# Autodesk Inventor assembly: HERA_NODE_ENCLOSURE_ASSEMBLY
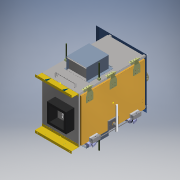
[picture p0: Inventor's stored thumbnail of the model, 180x180]
Saved by Autodesk Inventor 2018 (Build 220112000, 112)
## iProperties
Created: 2018-10-02
Part Number: HERA_NODE_ENCLOSURE_ASSEMBLY
Document SubType Name: Assembly
Designer: Francois
Mass: 169996 g
Surface Area: 258850 cm^2
Volume: 23149 cm^3
Density: 7.34355 g/cm^3
Author: Francois
## Documents named in this file (29)
- D:\ITC\DRAWINGS\SKA PROJECT\HERA NODE\HERA NODE 2018 TENDER SUBMISIONS\ASSEMBLY\HERA_NODE_ENCLOSURE_ASSEMBLY.iam
- D:\ITC\DRAWINGS\SKA PROJECT\HERA NODE\HERA NODE 2018 TENDER SUBMISIONS\PARTS\HERA_NODE_BOTTOM_PLATE.ipt
- D:\ITC\DRAWINGS\SKA PROJECT\HERA NODE\HERA NODE 2018 TENDER SUBMISIONS\PARTS\HERA_NODE_LEFT_SIDE_PLATE.ipt
- D:\ITC\DRAWINGS\SKA PROJECT\HERA NODE\HERA NODE 2018 TENDER SUBMISIONS\PARTS\HERA_NODE_RIGHT_SIDE_PLATE.ipt
- D:\ITC\DRAWINGS\SKA PROJECT\HERA NODE\HERA NODE 2018 TENDER SUBMISIONS\PARTS\HERA_NODE_TOP_PLATE.ipt
- D:\ITC\DRAWINGS\SKA PROJECT\HERA NODE\HERA NODE 2018 TENDER SUBMISIONS\PARTS\HERA_NODE_BACK_PLATE.ipt
- D:\ITC\DRAWINGS\SKA PROJECT\HERA NODE\HERA NODE 2018 TENDER SUBMISIONS\ASSEMBLY\HERA_NODE_FOOTPLATE_ASSEMBLY.iam
- D:\ITC\DRAWINGS\SKA PROJECT\HERA NODE\HERA NODE 2018 TENDER SUBMISIONS\ASSEMBLY\HERA_NODE_DOOR_ASSEMBLY.iam
- D:\ITC\DRAWINGS\SKA PROJECT\HERA NODE\HERA NODE 2018 TENDER SUBMISIONS\PARTS\FILTER PLATES\FILTER_PLATE_RP.ipt
- D:\ITC\DRAWINGS\SKA PROJECT\HERA NODE\HERA NODE 2018 TENDER SUBMISIONS\PARTS\FILTER PLATES\FILTER_PLATE_LP.ipt
- D:\ITC\DRAWINGS\SKA PROJECT\HERA NODE\HERA NODE 2018 TENDER SUBMISIONS\PARTS\HINGES\HINGE_ASSEMBLY.iam
- D:\ITC\DRAWINGS\SKA PROJECT\HERA NODE\HERA NODE 2018 TENDER SUBMISIONS\PARTS\FILTER PLATES\FILTER_PANEL_COVER_RP.ipt
- D:\ITC\DRAWINGS\SKA PROJECT\HERA NODE\HERA NODE 2018 TENDER SUBMISIONS\PARTS\LIFTING LUGS\LIFTING_LUG_SUPPORT.ipt
- D:\ITC\DRAWINGS\SKA PROJECT\HERA NODE\HERA NODE 2018 TENDER SUBMISIONS\PARTS\ROOF_PANEL.ipt
- D:\ITC\DRAWINGS\SKA PROJECT\HERA NODE\HERA NODE 2018 TENDER SUBMISIONS\PARTS\LIFTING LUGS\CARRY_HANDLE_SUPPORT.ipt
- D:\ITC\DRAWINGS\SKA PROJECT\HERA NODE\HERA NODE 2018 TENDER SUBMISIONS\PARTS\LIFTING LUGS\CARRY_HANDLE.ipt
- D:\ITC\DRAWINGS\SKA PROJECT\HERA NODE\HERA NODE 2018 TENDER SUBMISIONS\PARTS\DOOR HANDLE\DOOR_LOCK_CATCH.ipt
- D:\ITC\DRAWINGS\SKA PROJECT\HERA NODE\HERA NODE 2018 TENDER SUBMISIONS\ASSEMBLY\PART 1.ipt
- D:\ITC\DRAWINGS\SKA PROJECT\HERA NODE\HERA NODE 2018 TENDER SUBMISIONS\PARTS\VENTS\HERA_NODE_TOP_BOTTOM_ATTENUVENT.ipt
- D:\ITC\DRAWINGS\SKA PROJECT\HERA NODE\HERA NODE 2018 TENDER SUBMISIONS\PARTS\DINRAIL\DIN Rail (TS) 35mm Wide v1.ipt
- D:\ITC\DRAWINGS\SKA PROJECT\HERA NODE\HERA NODE 2018 TENDER SUBMISIONS\PARTS\DINRAIL\DIN Rail (TS) 35mm Wide v1\TS35x7.5 mm H - 6.2 mm dia slot - 225 mm long.ipt
- D:\ITC\DRAWINGS\SKA PROJECT\HERA NODE\HERA NODE 2018 TENDER SUBMISIONS\PARTS\LIFTING LUGS\M10 EYEBOLT.ipt
- D:\ITC\DRAWINGS\SKA PROJECT\HERA NODE\HERA NODE 2018 TENDER SUBMISIONS\PARTS\ALLBRO DB BOX\ALBRO_DB_BOX.iam
- D:\ITC\DRAWINGS\INVENTOR LIBRARY\DOOR HANDLES\SKA EN ABSA DEUR\DOOR HANDLE.iam
- D:\ITC\DRAWINGS\SKA PROJECT\HERA NODE\HERA NODE 2018 TENDER SUBMISIONS\PARTS\16A POWER FILTER\FILTER ASSEMBLY.iam
- D:\ITC\DRAWINGS\SKA PROJECT\HERA NODE\HERA NODE 2018 TENDER SUBMISIONS\PARTS\HINGES\FILTER PLATE COVER HINGES\4-3-4 bullet hinge.ipt
- D:\ITC\DRAWINGS\SKA PROJECT\HERA NODE\HERA NODE 2018 TENDER SUBMISIONS\PARTS\U_BRACKETS.ipt
- D:\ITC\DRAWINGS\SKA PROJECT\HERA NODE\HERA NODE 2018 TENDER SUBMISIONS\PARTS\CABLE TIE DOWN BAR\CABLE_TIE_DOWN_ASSEMBLY.iam
- D:\ITC\DRAWINGS\SKA PROJECT\HERA NODE\HERA NODE 2018 TENDER SUBMISIONS\PARTS\WHIRLEY BIRD\WHIRLEY BIRD.iam
## Components (50 placed, 27 different names)
1. HERA_NODE_BOTTOM_PLATE:1 — Mate:2, Flush:3, Flush:4, Mate:4, Flush:7, Flush:8, Mate:7, Mate:8, Mate:53, Mate:55
2. HERA_NODE_LEFT_SIDE_PLATE:1 — Mate:4, Flush:7, Flush:8, Mate:6, Flush:10, Flush:11, Mate:13, Mate:14, Mate:15, Mate:27, Flush:21, Flush:23, Flush:24, Flush:30, Mate:43, Mate:44, Flush:36, Mate:66, Mate:67, Mate:68, Mate:72
3. HERA_NODE_RIGHT_SIDE_PLATE:1 — Mate:2, Flush:3, Flush:4, Mate:3, Flush:5, Flush:6, Flush:12, Flush:13, Flush:14, Mate:10, Mate:11, Mate:12, Mate:26, Flush:25, Flush:26, Flush:27, Flush:29, Mate:41, Flush:32, Mate:42, Mate:64, Mate:65, Mate:70, Mate:73
4. HERA_NODE_TOP_PLATE:1 — Mate:3, Flush:5, Flush:6, Mate:5, Flush:9, Mate:9, Flush:15, Mate:32, Mate:33, Mate:34, Mate:35, Mate:54
5. HERA_NODE_BACK_PLATE:1 — Mate:5, Mate:6, Flush:9, Flush:22, Flush:28, Flush:34, Flush:38, Mate:56, Mate:61, Mate:63
6. HERA_NODE_FOOTPLATE_ASSEMBLY:1 [sub-assembly] — Mate:7, Flush:10, Flush:11, Flush:35, Flush:37
7. HERA_NODE_FOOTPLATE_ASSEMBLY:2 [sub-assembly] — Mate:8, Flush:12, Flush:13, Flush:31, Flush:33
8. HERA_NODE_DOOR_ASSEMBLY:1 [sub-assembly] — Mate:9, Flush:14, Flush:15, Mate:22, Flush:16, Mate:23, Flush:18, Mate:24, Flush:20, Mate:62, Flush:43, Flush:44
9. FILTER_PLATE_RP:1 — Mate:10, Mate:11, Mate:12, Mate:28, Mate:29
10. FILTER_PLATE_LP:1 — Mate:13, Mate:14, Mate:15, Mate:30, Mate:31
11. HINGE_ASSEMBLY:1 [sub-assembly] — Mate:22, Flush:16, Flush:17, Flush:19, Mate:25, Flush:20
12. HINGE_ASSEMBLY:2 [sub-assembly] — Mate:23, Flush:17, Flush:18
13. HINGE_ASSEMBLY:3 [sub-assembly] — Mate:24, Flush:19, Mate:25
14. FILTER_PANEL_COVER_RP:1 — Mate:26, Mate:28, Mate:29, Flush:45, Flush:46, Mate:71, Flush:50, Flush:53
15. FILTER_PANEL_COVER_RP:2 — Mate:27, Mate:30, Mate:31, Flush:47, Flush:48, Mate:69, Flush:49, Flush:54
16. LIFTING_LUG_SUPPORT:1 — Mate:33, Flush:23, Flush:24, Mate:60
17. LIFTING_LUG_SUPPORT:2 — Mate:34, Flush:25, Flush:26, Mate:36, Mate:59
18. LIFTING_LUG_SUPPORT:3 — Mate:32, Flush:21, Flush:22, Mate:58
19. LIFTING_LUG_SUPPORT:4 — Mate:35, Flush:27, Flush:28, Mate:57
20. ROOF_PANEL:1 — Mate:36, Flush:29, Flush:30, Mate:74
21. CARRY_HANDLE_SUPPORT:1 — Mate:44, Flush:35, Flush:36, Mate:46
22. CARRY_HANDLE_SUPPORT:2 — Mate:43, Flush:37, Flush:38, Mate:45
23. CARRY_HANDLE_SUPPORT:3 — Mate:42, Flush:33, Flush:34, Mate:48
24. CARRY_HANDLE_SUPPORT:4 — Mate:41, Flush:31, Flush:32, Mate:47
25. CARRY_HANDLE:1 — Mate:48
26. CARRY_HANDLE:2 — Mate:47
27. CARRY_HANDLE:3 — Mate:45
28. CARRY_HANDLE:4 — Mate:46
29. DOOR_LOCK_CATCH:1
30. DOOR_LOCK_CATCH:2
31. PART 1:1 — Mate:53
32. HERA_NODE_TOP_BOTTOM_ATTENUVENT:1 — Mate:54
33. HERA_NODE_TOP_BOTTOM_ATTENUVENT:2 — Mate:55
34. TS35x7.5 mm H - 6.2 mm dia slot - 225 mm long:1 — Mate:56
35. M10 EYEBOLT:1 — Mate:59
36. M10 EYEBOLT:2 — Mate:57
37. M10 EYEBOLT:3 — Mate:60
38. M10 EYEBOLT:4 — Mate:58
39. ALBRO_DB_BOX:1 [sub-assembly] — Mate:61
40. DOOR HANDLE:2 [sub-assembly] — Mate:62, Flush:43, Flush:44
41. FILTER ASSEMBLY:1 [sub-assembly] — Mate:63
42. 4-3-4 bullet hinge:1 — Mate:64, Flush:45
43. 4-3-4 bullet hinge:2 — Mate:65, Flush:46
44. 4-3-4 bullet hinge:3 — Mate:66, Flush:47
45. 4-3-4 bullet hinge:4 — Mate:67, Flush:48
46. U_BRACKETS:1 — Mate:68, Mate:69, Flush:49, Flush:55
47. U_BRACKETS:2 — Mate:70, Mate:71, Flush:50, Flush:56
48. CABLE_TIE_DOWN_ASSEMBLY:1 [sub-assembly] — Mate:73, Flush:53, Flush:56
49. CABLE_TIE_DOWN_ASSEMBLY:2 [sub-assembly] — Mate:72, Flush:54, Flush:55
50. WHIRLEY BIRD:1 [sub-assembly] — Mate:74
## Relationships (107: Mate 59, Flush 48)
- Mate:2: HERA_NODE_BOTTOM_PLATE:1 ↔ HERA_NODE_RIGHT_SIDE_PLATE:1
- Flush:3: HERA_NODE_BOTTOM_PLATE:1 ↔ HERA_NODE_RIGHT_SIDE_PLATE:1
- Flush:4: HERA_NODE_BOTTOM_PLATE:1 ↔ HERA_NODE_RIGHT_SIDE_PLATE:1
- Mate:3: HERA_NODE_RIGHT_SIDE_PLATE:1 ↔ HERA_NODE_TOP_PLATE:1
- Flush:5: HERA_NODE_RIGHT_SIDE_PLATE:1 ↔ HERA_NODE_TOP_PLATE:1
- Flush:6: HERA_NODE_RIGHT_SIDE_PLATE:1 ↔ HERA_NODE_TOP_PLATE:1
- Mate:4: HERA_NODE_BOTTOM_PLATE:1 ↔ HERA_NODE_LEFT_SIDE_PLATE:1
- Flush:7: HERA_NODE_BOTTOM_PLATE:1 ↔ HERA_NODE_LEFT_SIDE_PLATE:1
- Flush:8: HERA_NODE_BOTTOM_PLATE:1 ↔ HERA_NODE_LEFT_SIDE_PLATE:1
- Mate:5: HERA_NODE_TOP_PLATE:1 ↔ HERA_NODE_BACK_PLATE:1
- Mate:6: HERA_NODE_LEFT_SIDE_PLATE:1 ↔ HERA_NODE_BACK_PLATE:1
- Flush:9: HERA_NODE_TOP_PLATE:1 ↔ HERA_NODE_BACK_PLATE:1
- Mate:7: HERA_NODE_BOTTOM_PLATE:1 ↔ HERA_NODE_FOOTPLATE_ASSEMBLY:1
- Flush:10: HERA_NODE_LEFT_SIDE_PLATE:1 ↔ HERA_NODE_FOOTPLATE_ASSEMBLY:1
- Flush:11: HERA_NODE_LEFT_SIDE_PLATE:1 ↔ HERA_NODE_FOOTPLATE_ASSEMBLY:1
- Mate:8: HERA_NODE_BOTTOM_PLATE:1 ↔ HERA_NODE_FOOTPLATE_ASSEMBLY:2
- Flush:12: HERA_NODE_RIGHT_SIDE_PLATE:1 ↔ HERA_NODE_FOOTPLATE_ASSEMBLY:2
- Flush:13: HERA_NODE_RIGHT_SIDE_PLATE:1 ↔ HERA_NODE_FOOTPLATE_ASSEMBLY:2
- Mate:9: HERA_NODE_TOP_PLATE:1 ↔ HERA_NODE_DOOR_ASSEMBLY:1
- Flush:14 (33.4 mm): HERA_NODE_RIGHT_SIDE_PLATE:1 ↔ HERA_NODE_DOOR_ASSEMBLY:1
- Flush:15 (18.4 mm): HERA_NODE_TOP_PLATE:1 ↔ HERA_NODE_DOOR_ASSEMBLY:1
- Mate:10: HERA_NODE_RIGHT_SIDE_PLATE:1 ↔ FILTER_PLATE_RP:1
- Mate:11 (-40 mm): HERA_NODE_RIGHT_SIDE_PLATE:1 ↔ FILTER_PLATE_RP:1
- Mate:12 (-40 mm): HERA_NODE_RIGHT_SIDE_PLATE:1 ↔ FILTER_PLATE_RP:1
- Mate:13: HERA_NODE_LEFT_SIDE_PLATE:1 ↔ FILTER_PLATE_LP:1
- Mate:14 (-40 mm): HERA_NODE_LEFT_SIDE_PLATE:1 ↔ FILTER_PLATE_LP:1
- Mate:15 (-40 mm): HERA_NODE_LEFT_SIDE_PLATE:1 ↔ FILTER_PLATE_LP:1
- Mate:22: HERA_NODE_DOOR_ASSEMBLY:1 ↔ HINGE_ASSEMBLY:1
- Flush:16 (100 mm): HERA_NODE_DOOR_ASSEMBLY:1 ↔ HINGE_ASSEMBLY:1
- Mate:23: HERA_NODE_DOOR_ASSEMBLY:1 ↔ HINGE_ASSEMBLY:2
- Flush:17: HINGE_ASSEMBLY:1 ↔ HINGE_ASSEMBLY:2
- Flush:18 (100 mm): HERA_NODE_DOOR_ASSEMBLY:1 ↔ HINGE_ASSEMBLY:2
- Mate:24: HERA_NODE_DOOR_ASSEMBLY:1 ↔ HINGE_ASSEMBLY:3
- Flush:19: HINGE_ASSEMBLY:1 ↔ HINGE_ASSEMBLY:3
- Mate:25 (344.1 mm): HINGE_ASSEMBLY:1 ↔ HINGE_ASSEMBLY:3
- Mate:26: HERA_NODE_RIGHT_SIDE_PLATE:1 ↔ FILTER_PANEL_COVER_RP:1
- Mate:27: HERA_NODE_LEFT_SIDE_PLATE:1 ↔ FILTER_PANEL_COVER_RP:2
- Mate:28 (5 mm): FILTER_PLATE_RP:1 ↔ FILTER_PANEL_COVER_RP:1
- Mate:29 (3 mm): FILTER_PLATE_RP:1 ↔ FILTER_PANEL_COVER_RP:1
- Mate:30 (5 mm): FILTER_PLATE_LP:1 ↔ FILTER_PANEL_COVER_RP:2
- Mate:31 (3 mm): FILTER_PLATE_LP:1 ↔ FILTER_PANEL_COVER_RP:2
- Flush:20 (721.5 mm): HERA_NODE_DOOR_ASSEMBLY:1 ↔ HINGE_ASSEMBLY:1
- Mate:32: HERA_NODE_TOP_PLATE:1 ↔ LIFTING_LUG_SUPPORT:3
- Flush:21 (7 mm): HERA_NODE_LEFT_SIDE_PLATE:1 ↔ LIFTING_LUG_SUPPORT:3
- Flush:22 (7 mm): HERA_NODE_BACK_PLATE:1 ↔ LIFTING_LUG_SUPPORT:3
- Mate:33: HERA_NODE_TOP_PLATE:1 ↔ LIFTING_LUG_SUPPORT:1
- Flush:23 (7 mm): HERA_NODE_LEFT_SIDE_PLATE:1 ↔ LIFTING_LUG_SUPPORT:1
- Flush:24 (7 mm): HERA_NODE_LEFT_SIDE_PLATE:1 ↔ LIFTING_LUG_SUPPORT:1
- Mate:34: HERA_NODE_TOP_PLATE:1 ↔ LIFTING_LUG_SUPPORT:2
- Flush:25 (7 mm): HERA_NODE_RIGHT_SIDE_PLATE:1 ↔ LIFTING_LUG_SUPPORT:2
- Flush:26 (7 mm): HERA_NODE_RIGHT_SIDE_PLATE:1 ↔ LIFTING_LUG_SUPPORT:2
- Mate:35: HERA_NODE_TOP_PLATE:1 ↔ LIFTING_LUG_SUPPORT:4
- Flush:27 (7 mm): HERA_NODE_RIGHT_SIDE_PLATE:1 ↔ LIFTING_LUG_SUPPORT:4
- Flush:28 (7 mm): HERA_NODE_BACK_PLATE:1 ↔ LIFTING_LUG_SUPPORT:4
- Mate:36: LIFTING_LUG_SUPPORT:2 ↔ ROOF_PANEL:1
- Flush:29 (-9.2545 mm): HERA_NODE_RIGHT_SIDE_PLATE:1 ↔ ROOF_PANEL:1
- Flush:30 (-9.2545 mm): HERA_NODE_LEFT_SIDE_PLATE:1 ↔ ROOF_PANEL:1
- Mate:41: HERA_NODE_RIGHT_SIDE_PLATE:1 ↔ CARRY_HANDLE_SUPPORT:4
- Flush:31 (600 mm): HERA_NODE_FOOTPLATE_ASSEMBLY:2 ↔ CARRY_HANDLE_SUPPORT:4
- Flush:32 (20 mm): HERA_NODE_RIGHT_SIDE_PLATE:1 ↔ CARRY_HANDLE_SUPPORT:4
- Mate:42: HERA_NODE_RIGHT_SIDE_PLATE:1 ↔ CARRY_HANDLE_SUPPORT:3
- Flush:33 (600 mm): HERA_NODE_FOOTPLATE_ASSEMBLY:2 ↔ CARRY_HANDLE_SUPPORT:3
- Flush:34 (20 mm): HERA_NODE_BACK_PLATE:1 ↔ CARRY_HANDLE_SUPPORT:3
- Mate:43: HERA_NODE_LEFT_SIDE_PLATE:1 ↔ CARRY_HANDLE_SUPPORT:2
- Mate:44: HERA_NODE_LEFT_SIDE_PLATE:1 ↔ CARRY_HANDLE_SUPPORT:1
- Flush:35 (600 mm): HERA_NODE_FOOTPLATE_ASSEMBLY:1 ↔ CARRY_HANDLE_SUPPORT:1
- Flush:36 (20 mm): HERA_NODE_LEFT_SIDE_PLATE:1 ↔ CARRY_HANDLE_SUPPORT:1
- Flush:37 (600 mm): HERA_NODE_FOOTPLATE_ASSEMBLY:1 ↔ CARRY_HANDLE_SUPPORT:2
- Flush:38 (20 mm): HERA_NODE_BACK_PLATE:1 ↔ CARRY_HANDLE_SUPPORT:2
- Mate:45: CARRY_HANDLE_SUPPORT:2 ↔ CARRY_HANDLE:3
- Mate:46: CARRY_HANDLE_SUPPORT:1 ↔ CARRY_HANDLE:4
- Mate:47: CARRY_HANDLE_SUPPORT:4 ↔ CARRY_HANDLE:2
- Mate:48: CARRY_HANDLE_SUPPORT:3 ↔ CARRY_HANDLE:1
- Mate:53: HERA_NODE_BOTTOM_PLATE:1 ↔ PART 1:1
- Mate:54: HERA_NODE_TOP_PLATE:1 ↔ HERA_NODE_TOP_BOTTOM_ATTENUVENT:1
- Mate:55: HERA_NODE_BOTTOM_PLATE:1 ↔ HERA_NODE_TOP_BOTTOM_ATTENUVENT:2
- Mate:56: HERA_NODE_BACK_PLATE:1 ↔ TS35x7.5 mm H - 6.2 mm dia slot - 225 mm long:1
- Mate:57: LIFTING_LUG_SUPPORT:4 ↔ M10 EYEBOLT:2
- Mate:58: LIFTING_LUG_SUPPORT:3 ↔ M10 EYEBOLT:4
- Mate:59: LIFTING_LUG_SUPPORT:2 ↔ M10 EYEBOLT:1
- Mate:60: LIFTING_LUG_SUPPORT:1 ↔ M10 EYEBOLT:3
- Mate:61: HERA_NODE_BACK_PLATE:1 ↔ ALBRO_DB_BOX:1
- Mate:62: HERA_NODE_DOOR_ASSEMBLY:1 ↔ DOOR HANDLE:2
- Flush:43 (160.159 mm): HERA_NODE_DOOR_ASSEMBLY:1 ↔ DOOR HANDLE:2
- Flush:44: HERA_NODE_DOOR_ASSEMBLY:1 ↔ DOOR HANDLE:2
- Mate:63: HERA_NODE_BACK_PLATE:1 ↔ FILTER ASSEMBLY:1
- Mate:64: HERA_NODE_RIGHT_SIDE_PLATE:1 ↔ 4-3-4 bullet hinge:1
- Mate:65: HERA_NODE_RIGHT_SIDE_PLATE:1 ↔ 4-3-4 bullet hinge:2
- Flush:45 (50 mm): FILTER_PANEL_COVER_RP:1 ↔ 4-3-4 bullet hinge:1
- Flush:46 (50 mm): FILTER_PANEL_COVER_RP:1 ↔ 4-3-4 bullet hinge:2
- Mate:66: HERA_NODE_LEFT_SIDE_PLATE:1 ↔ 4-3-4 bullet hinge:3
- Flush:47 (50 mm): FILTER_PANEL_COVER_RP:2 ↔ 4-3-4 bullet hinge:3
- Mate:67: HERA_NODE_LEFT_SIDE_PLATE:1 ↔ 4-3-4 bullet hinge:4
- Flush:48 (50 mm): FILTER_PANEL_COVER_RP:2 ↔ 4-3-4 bullet hinge:4
- Mate:68: HERA_NODE_LEFT_SIDE_PLATE:1 ↔ U_BRACKETS:1
- Mate:69 (1 mm): FILTER_PANEL_COVER_RP:2 ↔ U_BRACKETS:1
- Flush:49: FILTER_PANEL_COVER_RP:2 ↔ U_BRACKETS:1
- Mate:70: HERA_NODE_RIGHT_SIDE_PLATE:1 ↔ U_BRACKETS:2
- Mate:71 (1 mm): FILTER_PANEL_COVER_RP:1 ↔ U_BRACKETS:2
- Flush:50: FILTER_PANEL_COVER_RP:1 ↔ U_BRACKETS:2
- Mate:72: HERA_NODE_LEFT_SIDE_PLATE:1 ↔ CABLE_TIE_DOWN_ASSEMBLY:2
- Mate:73: HERA_NODE_RIGHT_SIDE_PLATE:1 ↔ CABLE_TIE_DOWN_ASSEMBLY:1
- Flush:53 (-250 mm): FILTER_PANEL_COVER_RP:1 ↔ CABLE_TIE_DOWN_ASSEMBLY:1
- Flush:54 (-250 mm): FILTER_PANEL_COVER_RP:2 ↔ CABLE_TIE_DOWN_ASSEMBLY:2
- Flush:55: U_BRACKETS:1 ↔ CABLE_TIE_DOWN_ASSEMBLY:2
- Flush:56: U_BRACKETS:2 ↔ CABLE_TIE_DOWN_ASSEMBLY:1
- Mate:74: ROOF_PANEL:1 ↔ WHIRLEY BIRD:1
